# Autodesk Inventor assembly: サーボモータ25kgcm
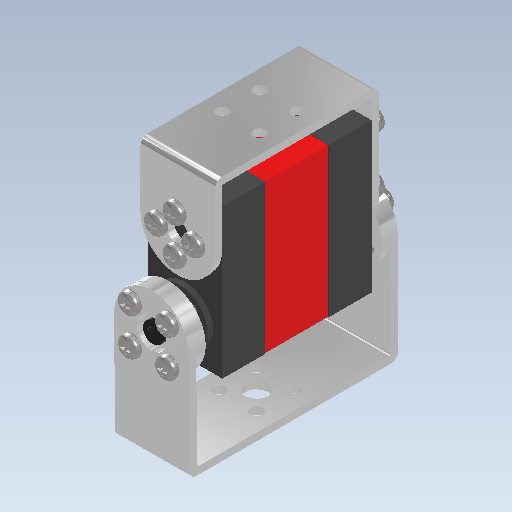
[picture p0: Inventor's stored thumbnail of the model, 512x512]
Saved by Autodesk Inventor 2021.2 (Build 252289000, 289)
## iProperties
Created: 2020-02-02
Part Number: サーボモータ25kgcm
Document SubType Name: Assembly
Designer: yuta2
Mass: 109.571 g
Surface Area: 175.932 cm^2
Volume: 40.5818 cm^3
Density: 2.7 g/cm^3
Author: yuta2
## Documents named in this file (8)
- C:\Users\Hagihara Yuya\Documents\GrabCAD\NHK2021\BasicParts\よく使う部品（萩原）\ServoMotor\Servo_DS3218MG\サーボモータ25kgcm.iam
- C:\Users\Hagihara Yuya\Documents\GrabCAD\NHK2021\BasicParts\よく使う部品（萩原）\ServoMotor\Servo_DS3218MG\サーボモーター25kgcmサーボモータ.ipt
- C:\Users\Hagihara Yuya\Documents\GrabCAD\NHK2021\BasicParts\よく使う部品（萩原）\ServoMotor\Servo_DS3218MG\サーボモータ25kgcmサーボホーン1.ipt
- C:\Users\Hagihara Yuya\Documents\GrabCAD\NHK2021\BasicParts\よく使う部品（萩原）\ServoMotor\Servo_DS3218MG\サーボモーター25kgcmサーボホーン2.ipt
- C:\Users\Hagihara Yuya\Documents\GrabCAD\NHK2021\BasicParts\よく使う部品（萩原）\ServoMotor\Servo_DS3218MG\サーボモーター25kgcmサーボホーン3.ipt
- C:\Users\Hagihara Yuya\Documents\GrabCAD\NHK2021\BasicParts\よく使う部品（萩原）\ServoMotor\Servo_DS3218MG\サーボモータ25kgcmサーボホーン4.ipt
- C:\Users\Hagihara Yuya\Documents\GrabCAD\NHK2021\Content Center Files\R2021\ja-JP\なべネジ\なべネジ - M3 x 6.ipt
- C:\Users\Hagihara Yuya\Documents\GrabCAD\NHK2021\Content Center Files\R2021\ja-JP\六角穴付きボルト\六角穴付きボルト - M3 × 5 - 0.5.ipt
## Components (24 placed, 7 different names)
1. サーボモーター25kgcmサーボモータ:1 — 回転:1, 回転:2, 回転:6, 回転:7, 回転:8, 回転:9
2. サーボモータ25kgcmサーボホーン4:1 — 回転:1, 回転:5
3. サーボモータ25kgcmサーボホーン1:2 — 回転:2, 回転:3, 回転:4, フラッシュ:39, メイト:37, フラッシュ:40
4. サーボモーター25kgcmサーボホーン2:1 — 回転:3, 回転:4, 回転:5, メイト:17, メイト:18, メイト:19, メイト:20, メイト:21, メイト:22, メイト:23, メイト:24, メイト:25, メイト:26, メイト:27, メイト:28, メイト:29, メイト:30, メイト:31, メイト:32, メイト:33, メイト:34, メイト:35, メイト:36
5. サーボモーター25kgcmサーボホーン3:1 — 回転:6, 回転:7, 回転:8, 回転:9, メイト:1, メイト:2, メイト:3, メイト:4, メイト:5, メイト:6, メイト:7, メイト:8, メイト:9, メイト:10, メイト:11, メイト:12, メイト:13, メイト:14, メイト:15, メイト:16
6. なべネジ M3 x 6:1 — メイト:1, メイト:2
7. なべネジ M3 x 6:2 — メイト:3, メイト:4
8. なべネジ M3 x 6:3 — メイト:5, メイト:6
9. なべネジ M3 x 6:4 — メイト:7, メイト:8
10. なべネジ M3 x 6:5 — メイト:9, メイト:10
11. なべネジ M3 x 6:6 — メイト:11, メイト:12
12. なべネジ M3 x 6:7 — メイト:13, メイト:14
13. なべネジ M3 x 6:8 — メイト:15, メイト:16
14. なべネジ M3 x 6:9 — メイト:17, メイト:18
15. なべネジ M3 x 6:10 — メイト:19, メイト:20
16. なべネジ M3 x 6:11 — メイト:21, メイト:22
17. なべネジ M3 x 6:12 — メイト:23, メイト:24
18. なべネジ M3 x 6:13 — メイト:25, メイト:26
19. なべネジ M3 x 6:14 — メイト:27, メイト:28
20. なべネジ M3 x 6:15 — メイト:29, メイト:30
21. なべネジ M3 x 6:16 — メイト:31, メイト:32
22. なべネジ M3 x 6:17 — メイト:33, メイト:34
23. なべネジ M3 x 6:18 — メイト:35, メイト:36
24. 六角穴付きボルト M3 x 5:1 — フラッシュ:39, メイト:37, フラッシュ:40
## Relationships (48: Mate 37, RevoluteJoint 9, Flush 2)
- 回転:1 [RevoluteJoint]: サーボモーター25kgcmサーボモータ:1 ↔ サーボモータ25kgcmサーボホーン4:1
- 回転:2 [RevoluteJoint]: サーボモーター25kgcmサーボモータ:1 ↔ サーボモータ25kgcmサーボホーン1:2
- 回転:3 [RevoluteJoint]: サーボモータ25kgcmサーボホーン1:2 ↔ サーボモーター25kgcmサーボホーン2:1
- 回転:4 [RevoluteJoint]: サーボモータ25kgcmサーボホーン1:2 ↔ サーボモーター25kgcmサーボホーン2:1
- 回転:5 [RevoluteJoint]: サーボモータ25kgcmサーボホーン4:1 ↔ サーボモーター25kgcmサーボホーン2:1
- 回転:6 [RevoluteJoint]: サーボモーター25kgcmサーボモータ:1 ↔ サーボモーター25kgcmサーボホーン3:1
- 回転:7 [RevoluteJoint]: サーボモーター25kgcmサーボモータ:1 ↔ サーボモーター25kgcmサーボホーン3:1
- 回転:8 [RevoluteJoint]: サーボモーター25kgcmサーボモータ:1 ↔ サーボモーター25kgcmサーボホーン3:1
- 回転:9 [RevoluteJoint]: サーボモーター25kgcmサーボモータ:1 ↔ サーボモーター25kgcmサーボホーン3:1
- メイト:1 [Mate]: サーボモーター25kgcmサーボホーン3:1 ↔ なべネジ M3 x 6:1
- メイト:2 [Mate]: サーボモーター25kgcmサーボホーン3:1 ↔ なべネジ M3 x 6:1
- メイト:3 [Mate]: サーボモーター25kgcmサーボホーン3:1 ↔ なべネジ M3 x 6:2
- メイト:4 [Mate]: サーボモーター25kgcmサーボホーン3:1 ↔ なべネジ M3 x 6:2
- メイト:5 [Mate]: サーボモーター25kgcmサーボホーン3:1 ↔ なべネジ M3 x 6:3
- メイト:6 [Mate]: サーボモーター25kgcmサーボホーン3:1 ↔ なべネジ M3 x 6:3
- メイト:7 [Mate]: サーボモーター25kgcmサーボホーン3:1 ↔ なべネジ M3 x 6:4
- メイト:8 [Mate]: サーボモーター25kgcmサーボホーン3:1 ↔ なべネジ M3 x 6:4
- メイト:9 [Mate]: サーボモーター25kgcmサーボホーン3:1 ↔ なべネジ M3 x 6:5
- メイト:10 [Mate]: サーボモーター25kgcmサーボホーン3:1 ↔ なべネジ M3 x 6:5
- メイト:11 [Mate]: サーボモーター25kgcmサーボホーン3:1 ↔ なべネジ M3 x 6:6
- メイト:12 [Mate]: サーボモーター25kgcmサーボホーン3:1 ↔ なべネジ M3 x 6:6
- メイト:13 [Mate]: サーボモーター25kgcmサーボホーン3:1 ↔ なべネジ M3 x 6:7
- メイト:14 [Mate]: サーボモーター25kgcmサーボホーン3:1 ↔ なべネジ M3 x 6:7
- メイト:15 [Mate]: サーボモーター25kgcmサーボホーン3:1 ↔ なべネジ M3 x 6:8
- メイト:16 [Mate]: サーボモーター25kgcmサーボホーン3:1 ↔ なべネジ M3 x 6:8
- メイト:17 [Mate]: サーボモーター25kgcmサーボホーン2:1 ↔ なべネジ M3 x 6:9
- メイト:18 [Mate]: サーボモーター25kgcmサーボホーン2:1 ↔ なべネジ M3 x 6:9
- メイト:19 [Mate]: サーボモーター25kgcmサーボホーン2:1 ↔ なべネジ M3 x 6:10
- メイト:20 [Mate]: サーボモーター25kgcmサーボホーン2:1 ↔ なべネジ M3 x 6:10
- メイト:21 [Mate]: サーボモーター25kgcmサーボホーン2:1 ↔ なべネジ M3 x 6:11
- メイト:22 [Mate]: サーボモーター25kgcmサーボホーン2:1 ↔ なべネジ M3 x 6:11
- メイト:23 [Mate]: サーボモーター25kgcmサーボホーン2:1 ↔ なべネジ M3 x 6:12
- メイト:24 [Mate]: サーボモーター25kgcmサーボホーン2:1 ↔ なべネジ M3 x 6:12
- メイト:25 [Mate]: サーボモーター25kgcmサーボホーン2:1 ↔ なべネジ M3 x 6:13
- メイト:26 [Mate]: サーボモーター25kgcmサーボホーン2:1 ↔ なべネジ M3 x 6:13
- メイト:27 [Mate]: サーボモーター25kgcmサーボホーン2:1 ↔ なべネジ M3 x 6:14
- メイト:28 [Mate]: サーボモーター25kgcmサーボホーン2:1 ↔ なべネジ M3 x 6:14
- メイト:29 [Mate]: サーボモーター25kgcmサーボホーン2:1 ↔ なべネジ M3 x 6:15
- メイト:30 [Mate]: サーボモーター25kgcmサーボホーン2:1 ↔ なべネジ M3 x 6:15
- メイト:31 [Mate]: サーボモーター25kgcmサーボホーン2:1 ↔ なべネジ M3 x 6:16
- メイト:32 [Mate]: サーボモーター25kgcmサーボホーン2:1 ↔ なべネジ M3 x 6:16
- メイト:33 [Mate]: サーボモーター25kgcmサーボホーン2:1 ↔ なべネジ M3 x 6:17
- メイト:34 [Mate]: サーボモーター25kgcmサーボホーン2:1 ↔ なべネジ M3 x 6:17
- メイト:35 [Mate]: サーボモーター25kgcmサーボホーン2:1 ↔ なべネジ M3 x 6:18
- メイト:36 [Mate]: サーボモーター25kgcmサーボホーン2:1 ↔ なべネジ M3 x 6:18
- フラッシュ:39 [Flush]: サーボモータ25kgcmサーボホーン1:2 ↔ 六角穴付きボルト M3 x 5:1
- メイト:37 [Mate]: サーボモータ25kgcmサーボホーン1:2 ↔ 六角穴付きボルト M3 x 5:1
- フラッシュ:40 [Flush]: サーボモータ25kgcmサーボホーン1:2 ↔ 六角穴付きボルト M3 x 5:1
